# Autodesk Inventor assembly: Jar Jar
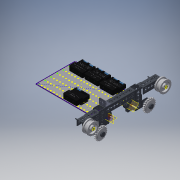
[picture p0: Inventor's stored thumbnail of the model, 180x180]
Saved by Autodesk Inventor 2016 (Build 200138000, 138)
## iProperties
Created: 2015-12-13
Part Number: Jar Jar
Document SubType Name: Assembly
Designer: tbloo
Author: tbloo
## Documents named in this file (16)
- C:\Users\TimB\Documents\GitHub\phi_robotics\3d-models\FTC_Tetrix_KOP_Block_Party\Tim Bloot Designs\JAr JaR Bot\Jar Jar.iam
- C:\Users\TimB\Documents\GitHub\phi_robotics\3d-models\FTC_Tetrix_KOP_Block_Party\Tim Bloot Designs\Base Plate.ipt
- C:\Users\TimB\Documents\GitHub\phi_robotics\3d-models\FTC_Tetrix_KOP_Block_Party\Tetrix_Kit_FTC\Autodesk Inventor Files\tetrix_c_channel-3.ipt
- C:\Users\TimB\Documents\GitHub\phi_robotics\3d-models\FTC_Tetrix_KOP_Block_Party\Tetrix_Kit_FTC\Autodesk Inventor Files\tetrix_c_channel-2.ipt
- C:\Users\TimB\Documents\GitHub\phi_robotics\3d-models\FTC_Tetrix_KOP_Block_Party\Tetrix_Kit_FTC\Autodesk Inventor Files\tetrix_motor_mount-old.ipt
- C:\Users\TimB\Documents\GitHub\phi_robotics\3d-models\FTC_Tetrix_KOP_Block_Party\Tetrix_Kit_FTC\Autodesk Inventor Files\tetrix_motor.iam
- C:\Users\TimB\Documents\GitHub\phi_robotics\3d-models\FTC_Tetrix_KOP_Block_Party\Tetrix_Kit_FTC\Autodesk Inventor Files\tetrix_bushing.ipt
- C:\Users\TimB\Documents\GitHub\phi_robotics\3d-models\FTC_Tetrix_KOP_Block_Party\Tim Bloot Designs\JAr JaR Bot\Tread Wheel Assembly.iam
- C:\Users\TimB\Documents\GitHub\phi_robotics\3d-models\FTC_Tetrix_KOP_Block_Party\Tetrix_Kit_FTC\Autodesk Inventor Files\tetrix_c_channel-5.ipt
- C:\Users\TimB\Documents\GitHub\phi_robotics\3d-models\FTC_Tetrix_KOP_Block_Party\Tetrix_Kit_FTC\Autodesk Inventor Files\tetrix_inside_corner_bracket.ipt
- C:\Users\TimB\Documents\GitHub\phi_robotics\3d-models\FTC_Tetrix_KOP_Block_Party\Tetrix_Kit_FTC\Autodesk Inventor Files\tetrix_motor_controller.ipt
- C:\Users\TimB\Documents\GitHub\phi_robotics\3d-models\FTC_Tetrix_KOP_Block_Party\Tetrix_Kit_FTC\Autodesk Inventor Files\tetrix_servo_controller.ipt
- C:\Users\TimB\Documents\GitHub\phi_robotics\3d-models\FTC_Tetrix_KOP_Block_Party\Tetrix_Kit_FTC\Autodesk Inventor Files\tetrix_c_channel-round.ipt
- C:\Users\TimB\Documents\GitHub\phi_robotics\3d-models\FTC_Tetrix_KOP_Block_Party\Tetrix_Kit_FTC\Autodesk Inventor Files\tetrix_c_channel-1.ipt
- C:\Users\TimB\Documents\GitHub\phi_robotics\3d-models\FTC_Tetrix_KOP_Block_Party\Tetrix_Kit_FTC\Autodesk Inventor Files\tetrix_angle-288 MM.ipt
- C:\Users\TimB\Documents\GitHub\phi_robotics\3d-models\FTC_Tetrix_KOP_Block_Party\Tim Bloot Designs\JAr JaR Bot\Tread Sproket Gear Assembly 2.iam
## Components (30 placed, 15 different names)
1. Base Plate:1 — Rigid:60, Rigid:61, Rigid:63, Rigid:85
2. tetrix_c_channel-3:4 — Rigid:55, Rigid:56, Rigid:76
3. tetrix_c_channel-2:13 — Rigid:64, Rigid:86
4. tetrix_c_channel-2:15
5. tetrix_c_channel-2:16
6. tetrix_motor_mount-old:6
7. tetrix_motor:5 [sub-assembly]
8. Tread Wheel Assembly:5 [sub-assembly]
9. Tread Wheel Assembly:6 [sub-assembly]
10. tetrix_c_channel-5:1 — Rigid:55
11. tetrix_c_channel-5:2 — Rigid:59
12. tetrix_inside_corner_bracket:2 — Rigid:56, Rigid:59
13. tetrix_motor_controller:1 — Rigid:61, Rigid:62
14. tetrix_motor_controller:2 — Rigid:60
15. tetrix_motor_controller:3 — Rigid:62
16. tetrix_servo_controller:1 — Rigid:63
17. tetrix_c_channel-round:1 — Rigid:64, Rigid:65
18. tetrix_c_channel-1:1 — Rigid:65, Rotational:33, Rotational:34
19. tetrix_bushing:13 — Rotational:33, Rotational:42
20. tetrix_bushing:14 — Rotational:34
21. tetrix_c_channel-2:18 — Rigid:75
22. tetrix_motor_mount-old:8 — Rotational:41
23. tetrix_c_channel-round:3
24. tetrix_c_channel-1:3
25. tetrix_bushing:17
26. tetrix_bushing:18 — Rotational:43
27. tetrix_angle-288 MM:2 — Rigid:75, Rigid:76, Rigid:85, Rigid:86
28. tetrix_motor:6 [sub-assembly] — Rotational:41
29. Tread Sproket Gear Assembly 2:1 [sub-assembly] — Rotational:42
30. Tread Sproket Gear Assembly 2:2 [sub-assembly] — Rotational:43
## Relationships (27: WeldJoint 17, RevoluteJoint 10)
- [WeldJoint]: tetrix_c_channel-2:13 ↔ tetrix_motor_mount-old:6
- [RevoluteJoint]: tetrix_motor_mount-old:6 ↔ tetrix_motor:5
- [RevoluteJoint]: tetrix_c_channel-2:15 ↔ Tread Wheel Assembly:5
- [RevoluteJoint]: tetrix_c_channel-2:16 ↔ Tread Wheel Assembly:6
- Rigid:55 [WeldJoint]: tetrix_c_channel-3:4 ↔ tetrix_c_channel-5:1
- Rigid:56 [WeldJoint]: tetrix_c_channel-3:4 ↔ tetrix_inside_corner_bracket:2
- Rigid:59 [WeldJoint]: tetrix_c_channel-5:2 ↔ tetrix_inside_corner_bracket:2
- Rigid:60 [WeldJoint]: Base Plate:1 ↔ tetrix_motor_controller:2
- Rigid:61 [WeldJoint]: Base Plate:1 ↔ tetrix_motor_controller:1
- Rigid:62 [WeldJoint]: tetrix_motor_controller:1 ↔ tetrix_motor_controller:3
- Rigid:63 [WeldJoint]: Base Plate:1 ↔ tetrix_servo_controller:1
- Rigid:64 [WeldJoint]: tetrix_c_channel-2:13 ↔ tetrix_c_channel-round:1
- Rigid:65 [WeldJoint]: tetrix_c_channel-round:1 ↔ tetrix_c_channel-1:1
- Rotational:33 [RevoluteJoint]: tetrix_c_channel-1:1 ↔ tetrix_bushing:13
- Rotational:34 [RevoluteJoint]: tetrix_c_channel-1:1 ↔ tetrix_bushing:14
- [WeldJoint]: tetrix_c_channel-2:18 ↔ tetrix_motor_mount-old:8
- [WeldJoint]: tetrix_c_channel-2:18 ↔ tetrix_c_channel-round:3
- [WeldJoint]: tetrix_c_channel-round:3 ↔ tetrix_c_channel-1:3
- [RevoluteJoint]: tetrix_c_channel-1:3 ↔ tetrix_bushing:17
- [RevoluteJoint]: tetrix_c_channel-1:3 ↔ tetrix_bushing:18
- Rigid:75 [WeldJoint]: tetrix_c_channel-2:18 ↔ tetrix_angle-288 MM:2
- Rigid:76 [WeldJoint]: tetrix_c_channel-3:4 ↔ tetrix_angle-288 MM:2
- Rotational:41 [RevoluteJoint]: tetrix_motor_mount-old:8 ↔ tetrix_motor:6
- Rotational:42 [RevoluteJoint]: tetrix_bushing:13 ↔ Tread Sproket Gear Assembly 2:1
- Rotational:43 [RevoluteJoint]: tetrix_bushing:18 ↔ Tread Sproket Gear Assembly 2:2
- Rigid:85 [WeldJoint]: Base Plate:1 ↔ tetrix_angle-288 MM:2
- Rigid:86 [WeldJoint]: tetrix_c_channel-2:13 ↔ tetrix_angle-288 MM:2
## Named parameters: d112_d58_d39 = 0 mm, d113_d59_d40 = -5.431137 deg, d114_d60_d41 = 0 mm, d115_d61_d42 = 0.840635 deg, d116_d65_d11 = 0 mm, d122_d71_d21 = 0 mm, d123_d72_d22 = -45.624239 deg, d153_d150_d116_d65_d11 = 0 mm, d154_d143_d137 = 0 mm, d155_d144_d138 = 0 mm, d156_d145_d139 = 0 mm, d157_d146_d140 = 0 deg, d158_d147_d141 = 0 mm, d159_d148_d142 = 0 deg
